# Autodesk Inventor assembly: Vaccuum_Assembly
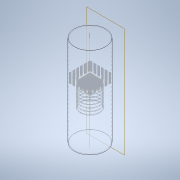
[picture p0: Inventor's stored thumbnail of the model, 180x180]
Saved by Autodesk Inventor 2021 (Build 250183000, 183)
## iProperties
Created: 2020-07-23
Part Number: Vaccuum_Assembly
Document SubType Name: Assembly
Designer: aydan
Author: aydan
## Documents named in this file (3)
- C:\Users\aydan\Documents\Inventor\Garcia_Lab\Vaccuum_Assembly.iam
- C:\Users\aydan\Documents\Inventor\Garcia_Lab\Chamber.ipt
- C:\Users\aydan\Documents\Inventor\Garcia_Lab\Final_Assembly.iam
## Components (2 placed, 2 different names)
1. Chamber:1 — Tangent:1, Mate:1, Mate:2
2. Final_Assembly:1 [sub-assembly] — Mate:2, Mate:3
## Relationships (5: Mate 3, Angle 1, Tangent 1)
- Angle:1 (0 deg)
- Tangent:1: Chamber:1
- Mate:1: Chamber:1
- Mate:2 (100 mm): Chamber:1 ↔ Final_Assembly:1
- Mate:3: Final_Assembly:1
